# Autodesk Inventor assembly: birdeye_elbowUnit_actuator
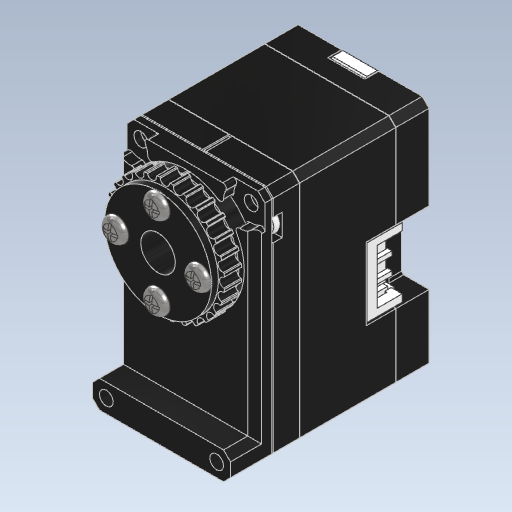
[picture p0: Inventor's stored thumbnail of the model, 512x512]
Saved by Autodesk Inventor 2024 (Build 280153000, 153)
## iProperties
Created: 2023-09-18
Part Number: birdeye_elbowUnit_actuator
Document SubType Name: Assembly
Designer: michi
Author: michi
## Documents named in this file (5)
- C:\Users\michi\OneDrive - Kyoto University\lab\6_SHINOBI\FUHGA4\Design_Mechanism\05_birdeye\birdeye_wristUnit\birdeye_wristUnit_actuator.iam
- C:\Users\michi\OneDrive - Kyoto University\lab\6_SHINOBI\FUHGA4\Design_Mechanism\00_devices\Dynamixel\X330\XL,XC-330.iam
- C:\Users\michi\OneDrive - Kyoto University\lab\6_SHINOBI\FUHGA4\Design_Mechanism\05_birdeye\birdeye__screw\Bolt_M2_10mm-selfTap_CSPPNSB-STU-TP2-10_203.ipt
- C:\Users\michi\OneDrive - Kyoto University\lab\6_SHINOBI\FUHGA4\Design_Mechanism\05_birdeye\birdeye_wristUnit\brideye_wristUnit_pully_active.ipt
- C:\Users\michi\OneDrive - Kyoto University\lab\6_SHINOBI\FUHGA4\Design_Mechanism\05_birdeye\birdeye_wristUnit\birdeye_wristUnit_spaser.ipt
## Components (7 placed, 4 different names)
1. XL,XC-330:1 [sub-assembly] — メイト:1, メイト:3, メイト:4, 回転:1, 回転:2
2. brideye_wristUnit_pully_active:1 — メイト:2, メイト:3, メイト:4, メイト:5
3. birdeye_wristUnit_spaser:1 — 回転:1, 回転:2
4. Bolt_M2_10mm-selfTap_CSPPNSB-STU-TP2-10_203:1 — メイト:1, メイト:2, メイト:5
5. Bolt_M2_10mm-selfTap_CSPPNSB-STU-TP2-10_203:2
6. Bolt_M2_10mm-selfTap_CSPPNSB-STU-TP2-10_203:3
7. Bolt_M2_10mm-selfTap_CSPPNSB-STU-TP2-10_203:4
## Component patterns: (4 elements, first: Bolt_M2_10mm-selfTap_CSPPNSB-STU-TP2-10_203:1)
## Relationships (7: Mate 5, RevoluteJoint 2)
- メイト:1 [Mate]: XL,XC-330:1 ↔ Bolt_M2_10mm-selfTap_CSPPNSB-STU-TP2-10_203:1
- メイト:2 [Mate]: brideye_wristUnit_pully_active:1 ↔ Bolt_M2_10mm-selfTap_CSPPNSB-STU-TP2-10_203:1
- メイト:3 [Mate]: XL,XC-330:1 ↔ brideye_wristUnit_pully_active:1
- メイト:4 [Mate]: XL,XC-330:1 ↔ brideye_wristUnit_pully_active:1
- メイト:5 [Mate]: brideye_wristUnit_pully_active:1 ↔ Bolt_M2_10mm-selfTap_CSPPNSB-STU-TP2-10_203:1
- 回転:1 [RevoluteJoint]: XL,XC-330:1 ↔ birdeye_wristUnit_spaser:1
- 回転:2 [RevoluteJoint]: XL,XC-330:1 ↔ birdeye_wristUnit_spaser:1
